# Autodesk Inventor assembly: gripper with jaws
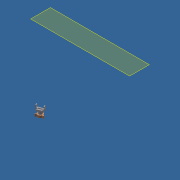
[picture p0: Inventor's stored thumbnail of the model, 180x180]
Saved by Autodesk Inventor 2012 (Build 160160000, 160)
## iProperties
Created: 2012-03-08
Part Number: gripper with jaws
Document SubType Name: Assembly
Designer: esv
Mass: 187059 g
Surface Area: 125343 cm^2
Volume: 160092 cm^3
Density: 1.16845 g/cm^3
Author: esv
## Documents named in this file (3)
- C:\Users\Ed\Documents\masters\CAD\Gripper\gripper with jaws.iam
- C:\Users\Ed\Documents\masters\CAD\Gripper\gripper.iam
- C:\Users\Ed\Documents\masters\CAD\Gripper\gripper jaw.ipt
## Components (3 placed, 2 different names)
1. gripper:2 [sub-assembly] — Flush:3, Mate:143, Mate:144
2. gripper jaw:1 — Mate:1, Flush:1, Flush:2
3. gripper jaw:2 — Mate:1, Flush:1, Flush:2, Flush:3, Mate:143, Mate:144
## Relationships (7: Mate 4, Flush 3)
- Mate:142
- Mate:1 (65.0875 mm): gripper jaw:1 ↔ gripper jaw:2
- Flush:1: gripper jaw:1 ↔ gripper jaw:2
- Flush:2: gripper jaw:1 ↔ gripper jaw:2
- Flush:3: gripper:2 ↔ gripper jaw:2
- Mate:143: gripper:2 ↔ gripper jaw:2
- Mate:144 (32.5438 mm): gripper:2 ↔ gripper jaw:2
